# Autodesk Inventor assembly: gantry
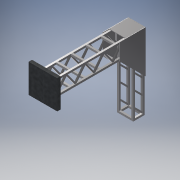
[picture p0: Inventor's stored thumbnail of the model, 180x180]
Saved by Autodesk Inventor 2016 (Build 200138000, 138)
## iProperties
Created: 2019-03-24
Part Number: gantry
Document SubType Name: Assembly
Designer: benja
Author: benja
## Documents named in this file (18)
- C:\Users\benja\Desktop\gantry.iam
- C:\Users\benja\Desktop\Short Horizontal for Truss.ipt
- C:\Users\benja\Desktop\Long post for truss.ipt
- C:\Users\benja\Desktop\Truss Structure.ipt
- C:\Users\benja\Desktop\cantilever long post.ipt
- C:\Users\benja\Desktop\Short Horizontal for Cantilever.ipt
- C:\Users\benja\Desktop\Long post for truss back.ipt
- C:\Users\benja\Desktop\Truss for cantilever.ipt
- C:\Users\benja\Desktop\back gusset.ipt
- C:\Users\benja\Desktop\exterior support.ipt
- C:\Users\benja\Desktop\side gusset.ipt
- C:\Users\benja\Desktop\top gusset.ipt
- C:\Users\benja\Desktop\base.ipt
- C:\Users\benja\Desktop\gantry\AIP\FEA\ctrju9xkw.fins
- C:\Users\benja\Desktop\gantry\AIP\FEA\ctrju9xkw.fsat
- C:\Users\benja\Desktop\gantry\AIP\FEA\ctrju9xkw.ftes
- C:\Users\benja\Desktop\gantry\AIP\FEA\ctrju9xls.fwiz
- C:\Users\benja\Desktop\gantry\AIP\FEA\ctrju9y0w.fmsh
## Components (51 placed, 12 different names)
1. Short Horizontal for Truss:1 — Flush:1, Mate:1, Mate:2, Mate:6, Mate:8, Flush:4, Flush:10, Mate:15, Flush:53, Flush:55, Mate:99, Flush:97
2. Short Horizontal for Truss:2 — Flush:2, Flush:3, Mate:3, Mate:4, Mate:5, Flush:11, Mate:11, Mate:13, Flush:56, Mate:78, Mate:79, Mate:80
3. Short Horizontal for Truss:3 — Flush:1, Flush:2, Mate:1, Mate:3, Mate:4, Mate:6, Flush:54, Flush:57, Flush:58, Mate:82, Flush:98
4. Short Horizontal for Truss:4 — Flush:3, Mate:2, Mate:5, Mate:7, Flush:8, Flush:12, Mate:28
5. Long post for truss:1 — Mate:8, Flush:4, Flush:10, Mate:14, Mate:16, Flush:13, Flush:14, Flush:59, Mate:91, Flush:89, Mate:94
6. Long post for truss:3 — Mate:7, Flush:8, Flush:11, Flush:12, Mate:12, Mate:13, Flush:16, Flush:17, Mate:17, Mate:18, Mate:24, Flush:26, Mate:25, Flush:27, Mate:26, Flush:28, Mate:27, Flush:29, Flush:60, Flush:80, Flush:81, Mate:93, Flush:88, Mate:95
7. Truss Structure:1 — Mate:11, Mate:12, Flush:60, Mate:78, Mate:79, Mate:80, Mate:81
8. Truss Structure:2 — Mate:14, Mate:15, Flush:59
9. Short Horizontal for Truss:5 — Flush:16, Flush:17, Mate:17
10. Short Horizontal for Truss:6 — Mate:18, Mate:81, Flush:80, Flush:81, Flush:83
11. Short Horizontal for Truss:7 — Mate:47, Flush:82, Flush:83, Mate:104
12. Short Horizontal for Truss:8 — Mate:16, Flush:13, Flush:14, Flush:52, Mate:48, Flush:77
13. Short Horizontal for Truss:9 — Mate:27, Flush:29, Mate:28, Mate:29
14. Short Horizontal for Truss:10 — Mate:26, Flush:28, Mate:29, Mate:30
15. Short Horizontal for Truss:11 — Mate:25, Flush:27, Mate:31
16. Short Horizontal for Truss:12 — Mate:33, Flush:87, Mate:82, Mate:83, Mate:103
17. Short Horizontal for Truss:13 — Mate:33, Mate:34, Flush:86, Mate:102
18. Short Horizontal for Truss:14 — Mate:35, Flush:84, Mate:100
19. Short Horizontal for Truss:15 — Mate:34, Mate:35, Flush:85, Mate:101
20. Short Horizontal for Truss:16 — Mate:24, Flush:26, Mate:30, Mate:31
21. cantilever long post:1 — Mate:37, Flush:30, Flush:31, Flush:39, Flush:42, Flush:46, Mate:44, Flush:76, Mate:92
22. cantilever long post:2 — Mate:39, Flush:36, Flush:37, Flush:44, Mate:49, Flush:63, Flush:65, Flush:67, Mate:75, Mate:76, Mate:77, Flush:92
23. cantilever long post:3 — Mate:38, Flush:34, Flush:35, Mate:41, Flush:40, Flush:41, Mate:46, Flush:69, Flush:71, Flush:73, Flush:75, Mate:71, Mate:72, Mate:73, Mate:74, Flush:90, Mate:96
24. cantilever long post:4 — Mate:36, Flush:32, Flush:33, Mate:40, Flush:38, Mate:45, Flush:48, Flush:49, Flush:50, Flush:52, Mate:48, Mate:70, Mate:90
25. Short Horizontal for Truss:17 — Mate:40, Flush:38, Flush:39, Flush:43, Mate:42, Flush:51
26. Short Horizontal for Truss:18 — Mate:38, Flush:34, Flush:35, Mate:39, Flush:36, Flush:37, Mate:105
27. Short Horizontal for Truss:19 — Mate:36, Mate:37, Flush:30, Flush:31, Flush:32, Flush:33, Flush:47
28. Short Horizontal for Truss:20 — Mate:41, Flush:40, Flush:41, Mate:43, Flush:45
29. Short Horizontal for Cantilever:1 — Mate:45, Flush:48, Flush:49, Mate:66, Mate:70
30. Short Horizontal for Cantilever:2 — Flush:50, Mate:46, Flush:51, Mate:47, Mate:68
31. Short Horizontal for Cantilever:3 — Flush:46, Flush:47, Mate:44, Flush:61, Mate:50, Mate:87
32. Short Horizontal for Cantilever:4 — Flush:42, Flush:43, Mate:42, Mate:43, Flush:44, Flush:45, Mate:67
33. Long post for truss back:1 — Flush:56, Flush:57, Flush:58, Flush:79, Mate:69, Flush:84, Flush:85, Flush:86, Flush:87, Mate:83, Mate:100, Mate:101, Mate:102, Mate:103
34. Long post for truss back:2 — Flush:53, Flush:54, Flush:55, Flush:78, Flush:82, Mate:104
35. Truss for cantilever:1 — Mate:49, Flush:61, Mate:50
36. Truss for cantilever:6 — Flush:67, Mate:76, Mate:86, Mate:89
37. Truss for cantilever:8 — Flush:63, Mate:75, Mate:84, Mate:87, Mate:88
38. Truss for cantilever:9 — Flush:65, Mate:77, Mate:85, Mate:88, Mate:89
39. Truss for cantilever:10 — Mate:66, Flush:69, Mate:105
40. Truss for cantilever:15 — Flush:75, Mate:73, Mate:86
41. Truss for cantilever:16 — Flush:71, Mate:71, Mate:84
42. Truss for cantilever:17 — Flush:73, Mate:72, Mate:85
43. Truss for cantilever:18 — Mate:67, Flush:76
44. Truss for cantilever:19 — Mate:68, Flush:77, Mate:74
45. back gusset:1 — Flush:78, Flush:79, Mate:69, Flush:91, Flush:93, Flush:94, Mate:98
46. exterior support:1 — Mate:90, Mate:91, Flush:89
47. exterior support:2 — Mate:92, Mate:93, Flush:88
48. side gusset:1 — Mate:94, Flush:90, Flush:91
49. side gusset:2 — Mate:95, Flush:92, Flush:93, Flush:95, Mate:97, Flush:96
50. top gusset:1 — Flush:94, Flush:95, Mate:96, Mate:97, Flush:96, Mate:98
51. base:1 — Mate:99, Flush:97, Flush:98
## Relationships (160: Mate 82, Flush 78)
- Flush:1: Short Horizontal for Truss:1 ↔ Short Horizontal for Truss:3
- Flush:2: Short Horizontal for Truss:2 ↔ Short Horizontal for Truss:3
- Flush:3: Short Horizontal for Truss:2 ↔ Short Horizontal for Truss:4
- Mate:1: Short Horizontal for Truss:1 ↔ Short Horizontal for Truss:3
- Mate:2: Short Horizontal for Truss:1 ↔ Short Horizontal for Truss:4
- Mate:3: Short Horizontal for Truss:2 ↔ Short Horizontal for Truss:3
- Mate:4: Short Horizontal for Truss:2 ↔ Short Horizontal for Truss:3
- Mate:5: Short Horizontal for Truss:2 ↔ Short Horizontal for Truss:4
- Mate:6: Short Horizontal for Truss:1 ↔ Short Horizontal for Truss:3
- Mate:7: Short Horizontal for Truss:4 ↔ Long post for truss:3
- Mate:8: Short Horizontal for Truss:1 ↔ Long post for truss:1
- Flush:4: Short Horizontal for Truss:1 ↔ Long post for truss:1
- Flush:8: Short Horizontal for Truss:4 ↔ Long post for truss:3
- Flush:10: Short Horizontal for Truss:1 ↔ Long post for truss:1
- Flush:11: Short Horizontal for Truss:2 ↔ Long post for truss:3
- Flush:12: Short Horizontal for Truss:4 ↔ Long post for truss:3
- Mate:11: Short Horizontal for Truss:2 ↔ Truss Structure:1
- Mate:12: Long post for truss:3 ↔ Truss Structure:1
- Mate:13: Short Horizontal for Truss:2 ↔ Long post for truss:3
- Mate:14: Long post for truss:1 ↔ Truss Structure:2
- Mate:15: Short Horizontal for Truss:1 ↔ Truss Structure:2
- Mate:16: Long post for truss:1 ↔ Short Horizontal for Truss:8
- Flush:13: Long post for truss:1 ↔ Short Horizontal for Truss:8
- Flush:14: Long post for truss:1 ↔ Short Horizontal for Truss:8
- Flush:16: Long post for truss:3 ↔ Short Horizontal for Truss:5
- Flush:17: Long post for truss:3 ↔ Short Horizontal for Truss:5
- Mate:17: Long post for truss:3 ↔ Short Horizontal for Truss:5
- Mate:18: Long post for truss:3 ↔ Short Horizontal for Truss:6
- Mate:24: Long post for truss:3 ↔ Short Horizontal for Truss:16
- Flush:26: Long post for truss:3 ↔ Short Horizontal for Truss:16
- Mate:25: Long post for truss:3 ↔ Short Horizontal for Truss:11
- Flush:27: Long post for truss:3 ↔ Short Horizontal for Truss:11
- Mate:26: Long post for truss:3 ↔ Short Horizontal for Truss:10
- Flush:28: Long post for truss:3 ↔ Short Horizontal for Truss:10
- Mate:27: Long post for truss:3 ↔ Short Horizontal for Truss:9
- Flush:29: Long post for truss:3 ↔ Short Horizontal for Truss:9
- Mate:28 (1468 mm): Short Horizontal for Truss:4 ↔ Short Horizontal for Truss:9
- Mate:29 (1368 mm): Short Horizontal for Truss:9 ↔ Short Horizontal for Truss:10
- Mate:30 (1368 mm): Short Horizontal for Truss:10 ↔ Short Horizontal for Truss:16
- Mate:31 (1368 mm): Short Horizontal for Truss:11 ↔ Short Horizontal for Truss:16
- Mate:33 (1368 mm): Short Horizontal for Truss:12 ↔ Short Horizontal for Truss:13
- Mate:34 (1368 mm): Short Horizontal for Truss:13 ↔ Short Horizontal for Truss:15
- Mate:35 (1368 mm): Short Horizontal for Truss:14 ↔ Short Horizontal for Truss:15
- Mate:36: cantilever long post:4 ↔ Short Horizontal for Truss:19
- Mate:37: cantilever long post:1 ↔ Short Horizontal for Truss:19
- Flush:30: cantilever long post:1 ↔ Short Horizontal for Truss:19
- Flush:31: cantilever long post:1 ↔ Short Horizontal for Truss:19
- Flush:32: cantilever long post:4 ↔ Short Horizontal for Truss:19
- Flush:33: cantilever long post:4 ↔ Short Horizontal for Truss:19
- Mate:38: cantilever long post:3 ↔ Short Horizontal for Truss:18
- Flush:34: cantilever long post:3 ↔ Short Horizontal for Truss:18
- Flush:35: cantilever long post:3 ↔ Short Horizontal for Truss:18
- Mate:39: cantilever long post:2 ↔ Short Horizontal for Truss:18
- Flush:36: cantilever long post:2 ↔ Short Horizontal for Truss:18
- Flush:37: cantilever long post:2 ↔ Short Horizontal for Truss:18
- Mate:40: cantilever long post:4 ↔ Short Horizontal for Truss:17
- Flush:38: cantilever long post:4 ↔ Short Horizontal for Truss:17
- Flush:39: cantilever long post:1 ↔ Short Horizontal for Truss:17
- Mate:41: cantilever long post:3 ↔ Short Horizontal for Truss:20
- Flush:40: cantilever long post:3 ↔ Short Horizontal for Truss:20
- Flush:41: cantilever long post:3 ↔ Short Horizontal for Truss:20
- Flush:42: cantilever long post:1 ↔ Short Horizontal for Cantilever:4
- Flush:43: Short Horizontal for Truss:17 ↔ Short Horizontal for Cantilever:4
- Mate:42: Short Horizontal for Truss:17 ↔ Short Horizontal for Cantilever:4
- Mate:43: Short Horizontal for Truss:20 ↔ Short Horizontal for Cantilever:4
- Flush:44: cantilever long post:2 ↔ Short Horizontal for Cantilever:4
- Flush:45: Short Horizontal for Truss:20 ↔ Short Horizontal for Cantilever:4
- Flush:46: cantilever long post:1 ↔ Short Horizontal for Cantilever:3
- Flush:47: Short Horizontal for Truss:19 ↔ Short Horizontal for Cantilever:3
- Mate:44: cantilever long post:1 ↔ Short Horizontal for Cantilever:3
- Mate:45: cantilever long post:4 ↔ Short Horizontal for Cantilever:1
- Flush:48: cantilever long post:4 ↔ Short Horizontal for Cantilever:1
- Flush:49: cantilever long post:4 ↔ Short Horizontal for Cantilever:1
- Flush:50: cantilever long post:4 ↔ Short Horizontal for Cantilever:2
- Mate:46: cantilever long post:3 ↔ Short Horizontal for Cantilever:2
- Flush:51: Short Horizontal for Truss:17 ↔ Short Horizontal for Cantilever:2
- Mate:47: Short Horizontal for Truss:7 ↔ Short Horizontal for Cantilever:2
- Flush:52: Short Horizontal for Truss:8 ↔ cantilever long post:4
- Mate:48: Short Horizontal for Truss:8 ↔ cantilever long post:4
- Flush:53: Short Horizontal for Truss:1 ↔ Long post for truss back:2
- Flush:54: Short Horizontal for Truss:3 ↔ Long post for truss back:2
- Flush:55: Short Horizontal for Truss:1 ↔ Long post for truss back:2
- Flush:56: Short Horizontal for Truss:2 ↔ Long post for truss back:1
- Flush:57: Short Horizontal for Truss:3 ↔ Long post for truss back:1
- Flush:58: Short Horizontal for Truss:3 ↔ Long post for truss back:1
- Flush:59 (30 mm): Long post for truss:1 ↔ Truss Structure:2
- Flush:60 (30 mm): Long post for truss:3 ↔ Truss Structure:1
- Mate:49: cantilever long post:2 ↔ Truss for cantilever:1
- Flush:61 (30 mm): Short Horizontal for Cantilever:3 ↔ Truss for cantilever:1
- Mate:50: Short Horizontal for Cantilever:3 ↔ Truss for cantilever:1
- Flush:63 (30 mm): cantilever long post:2 ↔ Truss for cantilever:8
- Flush:65 (30 mm): cantilever long post:2 ↔ Truss for cantilever:9
- Flush:67 (30 mm): cantilever long post:2 ↔ Truss for cantilever:6
- Mate:66: Short Horizontal for Cantilever:1 ↔ Truss for cantilever:10
- Flush:69 (30 mm): cantilever long post:3 ↔ Truss for cantilever:10
- Flush:71 (30 mm): cantilever long post:3 ↔ Truss for cantilever:16
- Flush:73 (30 mm): cantilever long post:3 ↔ Truss for cantilever:17
- Flush:75 (30 mm): cantilever long post:3 ↔ Truss for cantilever:15
- Mate:67: Short Horizontal for Cantilever:4 ↔ Truss for cantilever:18
- Flush:76 (30 mm): cantilever long post:1 ↔ Truss for cantilever:18
- Mate:68: Short Horizontal for Cantilever:2 ↔ Truss for cantilever:19
- Flush:77 (30 mm): Short Horizontal for Truss:8 ↔ Truss for cantilever:19
- Flush:78: Long post for truss back:2 ↔ back gusset:1
- Flush:79: Long post for truss back:1 ↔ back gusset:1
- Mate:69: Long post for truss back:1 ↔ back gusset:1
- Mate:70: cantilever long post:4 ↔ Short Horizontal for Cantilever:1
- Mate:71: cantilever long post:3 ↔ Truss for cantilever:16
- Mate:72: cantilever long post:3 ↔ Truss for cantilever:17
- Mate:73: cantilever long post:3 ↔ Truss for cantilever:15
- Mate:74: cantilever long post:3 ↔ Truss for cantilever:19
- Mate:75: cantilever long post:2 ↔ Truss for cantilever:8
- Mate:76: cantilever long post:2 ↔ Truss for cantilever:6
- Mate:77: cantilever long post:2 ↔ Truss for cantilever:9
- Mate:78: Short Horizontal for Truss:2 ↔ Truss Structure:1
- Mate:79: Short Horizontal for Truss:2 ↔ Truss Structure:1
- Mate:80: Short Horizontal for Truss:2 ↔ Truss Structure:1
- Mate:81: Truss Structure:1 ↔ Short Horizontal for Truss:6
- Flush:80: Long post for truss:3 ↔ Short Horizontal for Truss:6
- Flush:81: Long post for truss:3 ↔ Short Horizontal for Truss:6
- Flush:82: Short Horizontal for Truss:7 ↔ Long post for truss back:2
- Flush:83: Short Horizontal for Truss:6 ↔ Short Horizontal for Truss:7
- Flush:84: Short Horizontal for Truss:14 ↔ Long post for truss back:1
- Flush:85: Short Horizontal for Truss:15 ↔ Long post for truss back:1
- Flush:86: Short Horizontal for Truss:13 ↔ Long post for truss back:1
- Flush:87: Short Horizontal for Truss:12 ↔ Long post for truss back:1
- Mate:82 (1468 mm): Short Horizontal for Truss:3 ↔ Short Horizontal for Truss:12
- Mate:83: Short Horizontal for Truss:12 ↔ Long post for truss back:1
- Mate:84: Truss for cantilever:8 ↔ Truss for cantilever:16
- Mate:85: Truss for cantilever:9 ↔ Truss for cantilever:17
- Mate:86: Truss for cantilever:6 ↔ Truss for cantilever:15
- Mate:87 (1590.5025 mm): Short Horizontal for Cantilever:3 ↔ Truss for cantilever:8
- Mate:88 (1590.5025 mm): Truss for cantilever:8 ↔ Truss for cantilever:9
- Mate:89 (1590.5025 mm): Truss for cantilever:6 ↔ Truss for cantilever:9
- Mate:90: cantilever long post:4 ↔ exterior support:1
- Mate:91: Long post for truss:1 ↔ exterior support:1
- Mate:92: cantilever long post:1 ↔ exterior support:2
- Mate:93: Long post for truss:3 ↔ exterior support:2
- Flush:88: Long post for truss:3 ↔ exterior support:2
- Flush:89: Long post for truss:1 ↔ exterior support:1
- Mate:94: Long post for truss:1 ↔ side gusset:1
- Flush:90: cantilever long post:3 ↔ side gusset:1
- Flush:91: back gusset:1 ↔ side gusset:1
- Mate:95: Long post for truss:3 ↔ side gusset:2
- Flush:92: cantilever long post:2 ↔ side gusset:2
- Flush:93: back gusset:1 ↔ side gusset:2
- Flush:94: back gusset:1 ↔ top gusset:1
- Flush:95: side gusset:2 ↔ top gusset:1
- Mate:96: cantilever long post:3 ↔ top gusset:1
- Mate:97: side gusset:2 ↔ top gusset:1
- Flush:96: side gusset:2 ↔ top gusset:1
- Mate:98: back gusset:1 ↔ top gusset:1
- Mate:99: Short Horizontal for Truss:1 ↔ base:1
- Mate:100: Short Horizontal for Truss:14 ↔ Long post for truss back:1
- Mate:101: Short Horizontal for Truss:15 ↔ Long post for truss back:1
- Mate:102: Short Horizontal for Truss:13 ↔ Long post for truss back:1
- Mate:103: Short Horizontal for Truss:12 ↔ Long post for truss back:1
- Flush:97 (650 mm): Short Horizontal for Truss:1 ↔ base:1
- Flush:98 (650 mm): Short Horizontal for Truss:3 ↔ base:1
- Mate:104: Short Horizontal for Truss:7 ↔ Long post for truss back:2
- Mate:105: Short Horizontal for Truss:18 ↔ Truss for cantilever:10
